# Autodesk Inventor assembly: ПД Модуль 200х140х75
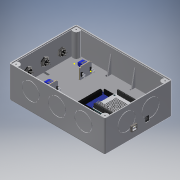
[picture p0: Inventor's stored thumbnail of the model, 180x180]
Saved by Autodesk Inventor 2019 (Build 230136000, 136)
## iProperties
Created: 2020-05-19
Part Number: ПД Модуль 200х140х75
Material: Типовые
Document SubType Name: Assembly
Designer: Surflay
Author: Surflay
## Documents named in this file (7)
- C:\Users\Surflay\Desktop\Университет\ПД\Модели\Газ (модуль)\ПД Модуль 200х140х75.iam
- C:\Users\Surflay\Desktop\Университет\ПД\Модели\Газ (модуль)\ПД Коробка 200х140х75.ipt
- C:\Users\Surflay\Desktop\Университет\ПД\Модели\Газ (модуль)\A_Arduino_Uno_Wifi_Shield.iam
- C:\Users\Surflay\Desktop\Университет\ПД\Модели\Газ (модуль)\3-pin\3-pin.iam
- C:\Users\Surflay\Desktop\Университет\ПД\Модели\Газ (модуль)\Arduino MEGA 2560 R3.ipt
- C:\Users\Surflay\Desktop\Университет\ПД\Модели\Газ (модуль)\Каркас.ipt
- C:\Users\Surflay\Desktop\Университет\ПД\Модели\Газ (модуль)\CAP.ipt
## Components (9 placed, 6 different names)
1. ПД Коробка 200х140х75:1 — Угол:2, Угол:3, Совмещение:6, Вставка:1, Вставка:2, Вставка:3, Совмещение:7, Совмещение:8
2. Arduino MEGA 2560 R3:1 — Угол:4, Угол:5, Совмещение:1, Совмещение:2, Совмещение:3, Совмещение:4, Совмещение:5, Касательность:1
3. A_Arduino_Uno_Wifi_Shield:1 [sub-assembly] — Угол:2, Угол:3, Угол:4, Угол:5, Совмещение:1, Совмещение:2, Совмещение:3
4. kls15-225-m12:1 [sub-assembly] — Вставка:3
5. kls15-225-m12:2 [sub-assembly] — Вставка:2
6. kls15-225-m12:3 [sub-assembly] — Вставка:1
7. Каркас:1 — Совмещение:4, Совмещение:5, Касательность:1, Совмещение:6, Угол:8, Совмещение:9
8. CAP:1 — Угол:8, Совмещение:7, Совмещение:8, Совмещение:9
9. CAP:2
## Component patterns: (2 elements, first: CAP:1)
## Relationships (18: Mate 9, Angle 5, Insert 3, Tangent 1)
- Угол:2 [Angle] (0 deg): ПД Коробка 200х140х75:1 ↔ A_Arduino_Uno_Wifi_Shield:1
- Угол:3 [Angle] (0 deg): ПД Коробка 200х140х75:1 ↔ A_Arduino_Uno_Wifi_Shield:1
- Угол:4 [Angle] (0 deg): Arduino MEGA 2560 R3:1 ↔ A_Arduino_Uno_Wifi_Shield:1
- Угол:5 [Angle] (90 deg): Arduino MEGA 2560 R3:1 ↔ A_Arduino_Uno_Wifi_Shield:1
- Совмещение:1 [Mate]: Arduino MEGA 2560 R3:1 ↔ A_Arduino_Uno_Wifi_Shield:1
- Совмещение:2 [Mate]: Arduino MEGA 2560 R3:1 ↔ A_Arduino_Uno_Wifi_Shield:1
- Совмещение:3 [Mate]: Arduino MEGA 2560 R3:1 ↔ A_Arduino_Uno_Wifi_Shield:1
- Совмещение:4 [Mate]: Arduino MEGA 2560 R3:1 ↔ Каркас:1
- Совмещение:5 [Mate]: Arduino MEGA 2560 R3:1 ↔ Каркас:1
- Касательность:1 [Tangent]: Arduino MEGA 2560 R3:1 ↔ Каркас:1
- Совмещение:6 [Mate]: ПД Коробка 200х140х75:1 ↔ Каркас:1
- Вставка:1 [Insert]: ПД Коробка 200х140х75:1 ↔ kls15-225-m12:3
- Вставка:2 [Insert]: ПД Коробка 200х140х75:1 ↔ kls15-225-m12:2
- Вставка:3 [Insert]: ПД Коробка 200х140х75:1 ↔ kls15-225-m12:1
- Угол:8 [Angle] (270 deg): Каркас:1 ↔ CAP:1
- Совмещение:7 [Mate] (20 mm): ПД Коробка 200х140х75:1 ↔ CAP:1
- Совмещение:8 [Mate] (40 mm): ПД Коробка 200х140х75:1 ↔ CAP:1
- Совмещение:9 [Mate]: Каркас:1 ↔ CAP:1
